# Autodesk Inventor assembly: MBD_Rl56
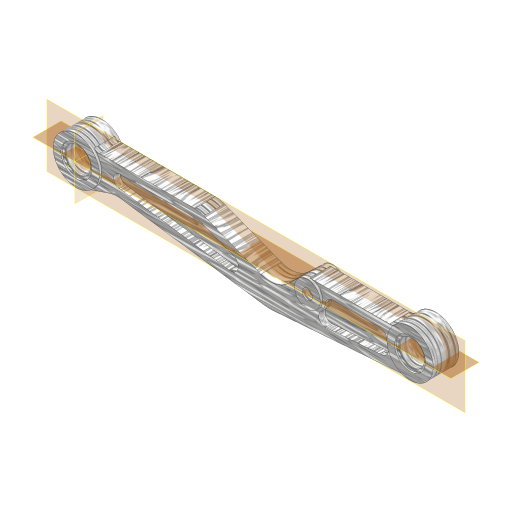
[picture p0: Inventor's stored thumbnail of the model, 512x512]
Saved by Autodesk Inventor 2023 (Build 270158000, 158)
## iProperties
Created: 2022-06-22
Part Number: MBD_Rl56
Document SubType Name: Assembly
Designer: BioRoLaT470S
Mass: 36.3774 g
Surface Area: 82.8753 cm^2
Volume: 12.9457 cm^3
Density: 2.81 g/cm^3
Author: BioRoLaT470S
## Documents named in this file (2)
- C:\Users\guanlunlu\Desktop\MBD_CORGI\CAD\MBD_Rl56.iam
- C:\Users\guanlunlu\Desktop\MBD_CORGI\R100_properties\組合檔_v4\I56_v2.ipt
## Components (1 placed, 1 different names)
1. I56_v2:1 — Mate:1, Mate:2, Flush:1
## Relationships (3: Mate 2, Flush 1)
- Mate:1: I56_v2:1
- Mate:2: I56_v2:1
- Flush:1: I56_v2:1
